# Autodesk Inventor assembly: base
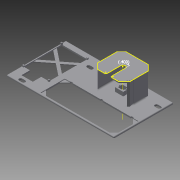
[picture p0: Inventor's stored thumbnail of the model, 180x180]
Saved by Autodesk Inventor 2014 SP2 (Build 180246200, 246)
## iProperties
Created: 2014-09-15
Part Number: base
Document SubType Name: Assembly
Designer: Rebecca
Author: Rebecca
## Documents named in this file (3)
- D:\Data\Autodesk\Projects\base.iam
- D:\Data\Autodesk\Projects\base 3a.ipt
- D:\Data\Autodesk\Projects\base 2b.ipt
## Components (2 placed, 2 different names)
1. base 3a:1 — Mate:1, Insert:1
2. base 2b:1 — Mate:2, Insert:1
## Relationships (3: Mate 2, Insert 1)
- Mate:1: base 3a:1
- Mate:2: base 2b:1
- Insert:1 (45.72 mm): base 3a:1 ↔ base 2b:1
